# Autodesk Inventor assembly: 200-60-DIFFERENTIAL-BAR-L-01
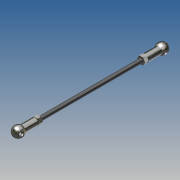
[picture p0: Inventor's stored thumbnail of the model, 180x180]
Saved by Autodesk Inventor 2018.2 (Build 222227000, 227)
## iProperties
Created: 2017-12-18
Part Number: 200-60-DIFFERENTIAL-BAR-L-01
Document SubType Name: Assembly
Designer: feesmrt
Author: feesmrt
## Documents named in this file (4)
- D:\Programmierung\FRANC0R\CAD\02-Rocker-Bogie-Robot\200-ROCKER-BOGIE\200-60-DIFFERENTIAL\200-60-DIFFERENTIAL-BAR-L-01.iam
- D:\Programmierung\FRANC0R\CAD\02-Rocker-Bogie-Robot\200-ROCKER-BOGIE\200-60-DIFFERENTIAL\200-60-DIFFERENTIAL-BAR-02.ipt
- D:\Programmierung\FRANC0R\CAD\02-Rocker-Bogie-Robot\900-COMPONENTS\900-70-ANGLE-JOINTS\900-70-ANGLE-JOINTS-DIN71802-M6-1.ipt
- D:\Programmierung\FRANC0R\CAD\02-Rocker-Bogie-Robot\900-COMPONENTS\900-41-NUTS\900-41-NUTS-ISO4033-M6.ipt
## Components (5 placed, 3 different names)
1. 200-60-DIFFERENTIAL-BAR-02:1 — Passend:1, Passend:2, Passend:3, Passend:4, Passend:5, Fluchtend:1, Passend:6, Passend:7
2. 900-70-ANGLE-JOINTS-DIN71802-M6-1:1 — Passend:1, Passend:3, Passend:5, Passend:8
3. 900-70-ANGLE-JOINTS-DIN71802-M6-1:2 — Passend:2, Passend:4, Fluchtend:1, Passend:9
4. 900-41-NUTS-ISO4033-M6:1 — Passend:6, Passend:8
5. 900-41-NUTS-ISO4033-M6:2 — Passend:7, Passend:9
## Relationships (10: Mate 9, Flush 1)
- Passend:1 [Mate]: 200-60-DIFFERENTIAL-BAR-02:1 ↔ 900-70-ANGLE-JOINTS-DIN71802-M6-1:1
- Passend:2 [Mate]: 200-60-DIFFERENTIAL-BAR-02:1 ↔ 900-70-ANGLE-JOINTS-DIN71802-M6-1:2
- Passend:3 [Mate] (-10 mm): 200-60-DIFFERENTIAL-BAR-02:1 ↔ 900-70-ANGLE-JOINTS-DIN71802-M6-1:1
- Passend:4 [Mate] (-10 mm): 200-60-DIFFERENTIAL-BAR-02:1 ↔ 900-70-ANGLE-JOINTS-DIN71802-M6-1:2
- Passend:5 [Mate]: 200-60-DIFFERENTIAL-BAR-02:1 ↔ 900-70-ANGLE-JOINTS-DIN71802-M6-1:1
- Fluchtend:1 [Flush]: 200-60-DIFFERENTIAL-BAR-02:1 ↔ 900-70-ANGLE-JOINTS-DIN71802-M6-1:2
- Passend:6 [Mate]: 200-60-DIFFERENTIAL-BAR-02:1 ↔ 900-41-NUTS-ISO4033-M6:1
- Passend:7 [Mate]: 200-60-DIFFERENTIAL-BAR-02:1 ↔ 900-41-NUTS-ISO4033-M6:2
- Passend:8 [Mate]: 900-70-ANGLE-JOINTS-DIN71802-M6-1:1 ↔ 900-41-NUTS-ISO4033-M6:1
- Passend:9 [Mate]: 900-70-ANGLE-JOINTS-DIN71802-M6-1:2 ↔ 900-41-NUTS-ISO4033-M6:2
